# Autodesk Inventor assembly: Drone_assembly
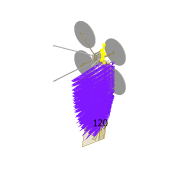
[picture p0: Inventor's stored thumbnail of the model, 180x180]
Saved by Autodesk Inventor 2022 (Build 260153000, 153)
## iProperties
Created: 2022-04-28
Part Number: Drone_assembly
Document SubType Name: Assembly
Designer: dell
Mass: 4396.41 g
Surface Area: 10173.4 cm^2
Volume: 3712.61 cm^3
Density: 1.18418 g/cm^3
Author: dell
## Documents named in this file (11)
- D:\xxxx\Uni\Part IV\MECHENG_700\Part_IV_project_CAD\Bird_skeleton_prototypes\Wing_drone_V1\Drone_assembly.iam
- D:\xxxx\Uni\Part IV\MECHENG_700\Part_IV_project_CAD\Bird_skeleton_prototypes\Wing_drone_V1\Drone_plate_1.ipt
- D:\xxxx\Uni\Part IV\MECHENG_700\Part_IV_project_CAD\Bird_skeleton_prototypes\Wing_drone_V1\Drone_rotor_arm_assembly.iam
- D:\xxxx\Uni\Part IV\MECHENG_700\Part_IV_project_CAD\Bird_skeleton_prototypes\Wing_drone_V1\Blade_simulator.ipt
- D:\xxxx\Uni\Part IV\MECHENG_700\Part_IV_project_CAD\Bird_skeleton_prototypes\Wing_drone_V1\Landing_leg\Landing_leg_assembly.iam
- D:\xxxx\Uni\Part IV\MECHENG_700\Part_IV_project_CAD\Bird_skeleton_prototypes\Wing_drone_V1\M3_spacer_27mm.ipt
- D:\xxxx\Uni\Part IV\MECHENG_700\Part_IV_project_CAD\Bird_skeleton_prototypes\Wing_drone_V1\Drone_plate_3.ipt
- D:\xxxx\Uni\Part IV\MECHENG_700\Part_IV_project_CAD\Bird_skeleton_prototypes\Wing_drone_V1\Foam_wing\Foam_wing.iam
- D:\xxxx\Uni\Part IV\MECHENG_700\Part_IV_project_CAD\Bird_skeleton_prototypes\Wing_drone_V1\Bird_wing_V2\Bird_wing_assembly.iam
- D:\xxxx\Uni\Part IV\MECHENG_700\Part_IV_project_CAD\Bird_skeleton_prototypes\Wing_drone_V1\Bird_wing_V2\Wing_shoulder\Shoulder_support_assembly.iam
- D:\xxxx\Uni\Part IV\MECHENG_700\Part_IV_project_CAD\Bird_skeleton_prototypes\Wing_drone_V1\Bird_wing_V2\Feather_0\Test_feather.ipt
## Components (24 placed, 10 different names)
1. Drone_plate_1:1 — Mate:3, Mate:12, Mate:14, Mate:16, Mate:17, Mate:19, Mate:20, Flush:1, Flush:2, Mate:22, Mate:23, Mate:24, Mate:25, Mate:26, Mate:65, Mate:66, Mate:67, Mate:79, Mate:80, Mate:81, Mate:82, Mate:83, Mate:84, Mate:85, Mate:86, Mate:87, Mate:90, Mate:100
2. Drone_rotor_arm_assembly:1 [sub-assembly] — Mate:3, Mate:4, Mate:5, Mate:21, Mate:23, Mate:24
3. Blade_simulator:1 — Mate:4, Mate:5
4. Drone_rotor_arm_assembly:2 [sub-assembly] — Mate:16, Mate:17, Mate:26
5. Blade_simulator:2
6. Drone_rotor_arm_assembly:3 [sub-assembly] — Mate:19, Mate:20, Mate:22
7. Blade_simulator:3
8. Drone_rotor_arm_assembly:4 [sub-assembly] — Mate:12, Mate:14, Mate:25
9. Blade_simulator:4
10. Drone_plate_1:2 — Mate:21, Flush:1, Flush:2, Mate:68, Mate:69, Mate:70, Mate:71, Mate:72, Mate:73, Mate:74, Mate:75, Mate:88, Mate:89, Mate:92, Mate:98, Mate:99
11. Landing_leg_assembly:1 [sub-assembly] — Mate:65, Mate:66, Mate:67
12. M3_spacer_27mm:1 — Mate:68, Mate:69
13. M3_spacer_27mm:2 — Mate:70, Mate:71
14. M3_spacer_27mm:3 — Mate:72, Mate:73, Mate:76
15. M3_spacer_27mm:4 — Mate:74, Mate:75, Mate:77, Mate:78
16. Drone_plate_3:1 — Mate:76, Mate:77, Mate:78
17. Landing_leg_assembly:2 [sub-assembly] — Mate:85, Mate:86, Mate:87
18. Landing_leg_assembly:3 [sub-assembly] — Mate:82, Mate:83, Mate:84
19. Landing_leg_assembly:4 [sub-assembly] — Mate:79, Mate:80, Mate:81
20. Foam_wing:1 [sub-assembly] — Mate:88, Mate:89, Mate:90
21. Bird_wing_assembly:1 [sub-assembly] — Mate:101, Mate:102, Mate:103, Mate:104
22. Shoulder_support_assembly:1 [sub-assembly] — Mate:92, Mate:98, Mate:99, Mate:100, Mate:101, Mate:102
23. Test_feather:3 — Mate:103
24. Test_feather:4 — Mate:104
## Relationships (57: Mate 55, Flush 2)
- Mate:3: Drone_plate_1:1 ↔ Drone_rotor_arm_assembly:1
- Mate:4: Drone_rotor_arm_assembly:1 ↔ Blade_simulator:1
- Mate:5: Drone_rotor_arm_assembly:1 ↔ Blade_simulator:1
- [Mate]: Drone_rotor_arm_assembly:2 ↔ Blade_simulator:2
- [Mate]: Drone_rotor_arm_assembly:2 ↔ Blade_simulator:2
- [Mate]: Drone_rotor_arm_assembly:3 ↔ Blade_simulator:3
- [Mate]: Drone_rotor_arm_assembly:3 ↔ Blade_simulator:3
- [Mate]: Drone_rotor_arm_assembly:4 ↔ Blade_simulator:4
- [Mate]: Drone_rotor_arm_assembly:4 ↔ Blade_simulator:4
- Mate:12: Drone_plate_1:1 ↔ Drone_rotor_arm_assembly:4
- Mate:14: Drone_plate_1:1 ↔ Drone_rotor_arm_assembly:4
- Mate:16: Drone_plate_1:1 ↔ Drone_rotor_arm_assembly:2
- Mate:17: Drone_plate_1:1 ↔ Drone_rotor_arm_assembly:2
- Mate:19: Drone_plate_1:1 ↔ Drone_rotor_arm_assembly:3
- Mate:20: Drone_plate_1:1 ↔ Drone_rotor_arm_assembly:3
- Mate:21: Drone_rotor_arm_assembly:1 ↔ Drone_plate_1:2
- Flush:1: Drone_plate_1:1 ↔ Drone_plate_1:2
- Flush:2: Drone_plate_1:1 ↔ Drone_plate_1:2
- Mate:22: Drone_plate_1:1 ↔ Drone_rotor_arm_assembly:3
- Mate:23: Drone_plate_1:1 ↔ Drone_rotor_arm_assembly:1
- Mate:24: Drone_plate_1:1 ↔ Drone_rotor_arm_assembly:1
- Mate:25: Drone_plate_1:1 ↔ Drone_rotor_arm_assembly:4
- Mate:26: Drone_plate_1:1 ↔ Drone_rotor_arm_assembly:2
- Mate:65: Drone_plate_1:1 ↔ Landing_leg_assembly:1
- Mate:66: Drone_plate_1:1 ↔ Landing_leg_assembly:1
- Mate:67: Drone_plate_1:1 ↔ Landing_leg_assembly:1
- Mate:68: Drone_plate_1:2 ↔ M3_spacer_27mm:1
- Mate:69: Drone_plate_1:2 ↔ M3_spacer_27mm:1
- Mate:70: Drone_plate_1:2 ↔ M3_spacer_27mm:2
- Mate:71: Drone_plate_1:2 ↔ M3_spacer_27mm:2
- Mate:72: Drone_plate_1:2 ↔ M3_spacer_27mm:3
- Mate:73: Drone_plate_1:2 ↔ M3_spacer_27mm:3
- Mate:74: Drone_plate_1:2 ↔ M3_spacer_27mm:4
- Mate:75: Drone_plate_1:2 ↔ M3_spacer_27mm:4
- Mate:76: M3_spacer_27mm:3 ↔ Drone_plate_3:1
- Mate:77: M3_spacer_27mm:4 ↔ Drone_plate_3:1
- Mate:78: M3_spacer_27mm:4 ↔ Drone_plate_3:1
- Mate:79: Drone_plate_1:1 ↔ Landing_leg_assembly:4
- Mate:80: Drone_plate_1:1 ↔ Landing_leg_assembly:4
- Mate:81: Drone_plate_1:1 ↔ Landing_leg_assembly:4
- Mate:82: Drone_plate_1:1 ↔ Landing_leg_assembly:3
- Mate:83: Drone_plate_1:1 ↔ Landing_leg_assembly:3
- Mate:84: Drone_plate_1:1 ↔ Landing_leg_assembly:3
- Mate:85: Drone_plate_1:1 ↔ Landing_leg_assembly:2
- Mate:86: Drone_plate_1:1 ↔ Landing_leg_assembly:2
- Mate:87: Drone_plate_1:1 ↔ Landing_leg_assembly:2
- Mate:88: Drone_plate_1:2 ↔ Foam_wing:1
- Mate:89: Drone_plate_1:2 ↔ Foam_wing:1
- Mate:90: Drone_plate_1:1 ↔ Foam_wing:1
- Mate:92: Drone_plate_1:2 ↔ Shoulder_support_assembly:1
- Mate:98: Drone_plate_1:2 ↔ Shoulder_support_assembly:1
- Mate:99: Drone_plate_1:2 ↔ Shoulder_support_assembly:1
- Mate:100: Drone_plate_1:1 ↔ Shoulder_support_assembly:1
- Mate:101: Bird_wing_assembly:1 ↔ Shoulder_support_assembly:1
- Mate:102: Bird_wing_assembly:1 ↔ Shoulder_support_assembly:1
- Mate:103: Bird_wing_assembly:1 ↔ Test_feather:3
- Mate:104: Bird_wing_assembly:1 ↔ Test_feather:4
## Named parameters: d44_d41 = 0 mm, d45_d43 = 0 mm, d46_d41 = 0 mm, d47_d43 = 0 mm, d48_d41 = 0 mm, d49_d43 = 0 mm
